# Autodesk Inventor assembly: Robot_Rev3
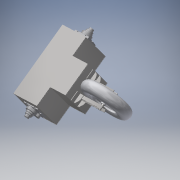
[picture p0: Inventor's stored thumbnail of the model, 180x180]
Saved by Autodesk Inventor 2017 (Build 210142000, 142)
## iProperties
Created: 2016-12-07
Part Number: Robot_Rev3
Document SubType Name: Assembly
Designer: Robert.Chapman
Mass: 35652.1 g
Surface Area: 18972.2 cm^2
Volume: 11102.4 cm^3
Density: 3.21122 g/cm^3
Author: Robert.Chapman
## Documents named in this file (15)
- C:\Users\Robert.Chapman\Documents\Robot_Rev3.iam
- C:\Users\Robert.Chapman\Documents\FrontPlow.ipt
- C:\Users\Robert.Chapman\Documents\LeftSide.ipt
- C:\Users\Robert.Chapman\Documents\LeftRightInner.ipt
- C:\Users\Robert.Chapman\Documents\LongTLeftRightOut.ipt
- C:\Users\Robert.Chapman\Documents\RearInnerTLeftRight.ipt
- C:\Users\Robert.Chapman\Documents\top_bottom_rev2.ipt
- C:\Users\Robert.Chapman\Documents\Rear.ipt
- C:\Users\Robert.Chapman\Downloads\NPC-T74.ipt
- C:\Users\Robert.Chapman\Documents\RearWheelMount.ipt
- C:\Users\Robert.Chapman\Documents\RearWheel.ipt
- C:\Users\Robert.Chapman\Documents\RearChannel.ipt
- C:\Users\Robert.Chapman\Documents\RearAxle.ipt
- C:\Users\Robert.Chapman\Documents\TopPlate.ipt
- C:\Users\Robert.Chapman\Documents\RearWheelMountLeft.ipt
## Components (21 placed, 14 different names)
1. FrontPlow:1 — Mate:65, Mate:67, Mate:86, Mate:126
2. LeftSide:1 — Mate:67, Mate:70, Mate:87, Mate:128
3. LeftSide:2 — Mate:65, Mate:68, Mate:90, Mate:91
4. LeftRightInner:1 — Mate:68, Mate:72
5. LeftRightInner:2 — Mate:70, Mate:85
6. LongTLeftRightOut:1 — Mate:72
7. LongTLeftRightOut:2 — Mate:85, Mate:89
8. RearInnerTLeftRight:2
9. top_bottom_rev2:1 — Mate:86, Mate:87, Mate:88
10. Rear:1 — Mate:88, Mate:89, Mate:97, Mate:98, Mate:102, Mate:127, Mate:141, Mate:142, Mate:143, Mate:145, Mate:146, Mate:148
11. NPC-T74:1
12. NPC-T74:2 — Mate:90, Mate:91
13. RearWheel:1 — Mate:109, Mate:110
14. RearChannel:1 — Mate:97, Mate:101, Mate:102, Mate:129, Mate:130, Mate:131, Mate:140, Mate:144
15. RearChannel:2 — Mate:98, Mate:101, Mate:107, Mate:108, Mate:110, Mate:117, Mate:118, Mate:119, Mate:120, Mate:121, Mate:122, Mate:125, Mate:139, Mate:147, Mate:149, Mate:150
16. RearAxle:1 — Mate:107, Mate:108, Mate:109, Mate:117, Mate:118, Mate:119, Mate:120, Mate:121, Mate:122, Mate:125, Mate:129, Mate:130, Mate:131, Mate:139, Mate:149, Mate:150
17. RearWheelMount:4
18. TopPlate:1 — Mate:126, Mate:127, Mate:128
19. RearWheelMount:6 — Mate:140, Mate:141, Mate:142
20. RearWheelMountLeft:1 — Mate:146, Mate:147, Mate:148
21. RearWheelMountLeft:2 — Mate:143, Mate:144, Mate:145
## Relationships (45: Mate 45)
- Mate:65: FrontPlow:1 ↔ LeftSide:2
- Mate:67: FrontPlow:1 ↔ LeftSide:1
- Mate:68: LeftSide:2 ↔ LeftRightInner:1
- Mate:70: LeftSide:1 ↔ LeftRightInner:2
- Mate:72: LeftRightInner:1 ↔ LongTLeftRightOut:1
- Mate:85: LeftRightInner:2 ↔ LongTLeftRightOut:2
- Mate:86: FrontPlow:1 ↔ top_bottom_rev2:1
- Mate:87: LeftSide:1 ↔ top_bottom_rev2:1
- Mate:88: top_bottom_rev2:1 ↔ Rear:1
- Mate:89: LongTLeftRightOut:2 ↔ Rear:1
- Mate:90: LeftSide:2 ↔ NPC-T74:2
- Mate:91: LeftSide:2 ↔ NPC-T74:2
- Mate:97: Rear:1 ↔ RearChannel:1
- Mate:98: Rear:1 ↔ RearChannel:2
- Mate:101 (101.6 mm): RearChannel:1 ↔ RearChannel:2
- Mate:102 (71.4375 mm): Rear:1 ↔ RearChannel:1
- Mate:107: RearChannel:2 ↔ RearAxle:1
- Mate:108 (25.4 mm): RearChannel:2 ↔ RearAxle:1
- Mate:109: RearWheel:1 ↔ RearAxle:1
- Mate:110 (12.7 mm): RearWheel:1 ↔ RearChannel:2
- Mate:117: RearChannel:2 ↔ RearAxle:1
- Mate:118: RearChannel:2 ↔ RearAxle:1
- Mate:119: RearChannel:2 ↔ RearAxle:1
- Mate:120: RearChannel:2 ↔ RearAxle:1
- Mate:121: RearChannel:2 ↔ RearAxle:1
- Mate:122: RearChannel:2 ↔ RearAxle:1
- Mate:125: RearChannel:2 ↔ RearAxle:1
- Mate:126: FrontPlow:1 ↔ TopPlate:1
- Mate:127: Rear:1 ↔ TopPlate:1
- Mate:128: LeftSide:1 ↔ TopPlate:1
- Mate:129: RearChannel:1 ↔ RearAxle:1
- Mate:130: RearChannel:1 ↔ RearAxle:1
- Mate:131: RearChannel:1 ↔ RearAxle:1
- Mate:139: RearChannel:2 ↔ RearAxle:1
- Mate:140: RearChannel:1 ↔ RearWheelMount:6
- Mate:141: Rear:1 ↔ RearWheelMount:6
- Mate:142: Rear:1 ↔ RearWheelMount:6
- Mate:143: Rear:1 ↔ RearWheelMountLeft:2
- Mate:144: RearChannel:1 ↔ RearWheelMountLeft:2
- Mate:145: Rear:1 ↔ RearWheelMountLeft:2
- Mate:146: Rear:1 ↔ RearWheelMountLeft:1
- Mate:147: RearChannel:2 ↔ RearWheelMountLeft:1
- Mate:148: Rear:1 ↔ RearWheelMountLeft:1
- Mate:149: RearChannel:2 ↔ RearAxle:1
- Mate:150: RearChannel:2 ↔ RearAxle:1
